# Autodesk Inventor assembly: KS-14_SLow_replace
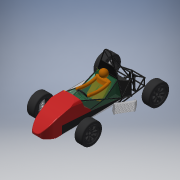
[picture p0: Inventor's stored thumbnail of the model, 180x180]
Saved by Autodesk Inventor 2018.1 (Build 221171000, 171)
## iProperties
Created: 2017-11-01
Part Number: KS-14_SLow_replace
Material: 一般
Document SubType Name: Assembly
Designer: kuwano
Author: kuwano
## Documents named in this file (2)
- D:\kuwano\Documents\Inventor\KITformula\KS-15_Aero_CAD\ks-14_slow\KS-14_SLow_replace.iam
- D:\kuwano\Documents\Inventor\KITformula\KS-15_Aero_CAD\ks-14_slow\KS-14_SLow.iam
## Components (1 placed, 1 different names)
1. KS-14_SLow:1 [sub-assembly] — メイト:1, フラッシュ:1, 正接:1
## Relationships (3: Mate 1, Flush 1, Tangent 1)
- メイト:1 [Mate]: KS-14_SLow:1
- フラッシュ:1 [Flush]: KS-14_SLow:1
- 正接:1 [Tangent]: KS-14_SLow:1
